# Autodesk Inventor assembly: iDISCO-Sampleholder-Assembly
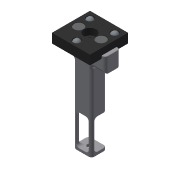
[picture p0: Inventor's stored thumbnail of the model, 180x180]
Saved by Autodesk Inventor 2016 (Build 200138000, 138)
## iProperties
Created: 2019-02-05
Part Number: iDISCO-Sampleholder-Assembly
Document SubType Name: Assembly
Designer: voigt
Author: voigt
## Documents named in this file (3)
- D:\Microscope_Design\CAD_Files\mesoSPIM_design_V4\mesoSPIM_design\mesoSPIM\sample_handling\IDISCO-Sampleholder\iDISCO-Sampleholder-Assembly.iam
- D:\Microscope_Design\CAD_Files\mesoSPIM_design_V4\mesoSPIM_design\library\Thorlabs\kinematic_bases\KBT25_M.ipt
- D:\Microscope_Design\CAD_Files\mesoSPIM_design_V4\mesoSPIM_design\mesoSPIM\sample_handling\IDISCO-Sampleholder\IDISCO-Sampleholder-12mm-60mm_V2_Sascha.ipt
## Components (2 placed, 2 different names)
1. KBT25_M:1 — Mate:1, Angle:1, Mate:2
2. IDISCO-Sampleholder-12mm-60mm_V2_Sascha:1 — Mate:1, Angle:1, Mate:2
## Relationships (3: Mate 2, Angle 1)
- Mate:1: KBT25_M:1 ↔ IDISCO-Sampleholder-12mm-60mm_V2_Sascha:1
- Angle:1 (90 deg): KBT25_M:1 ↔ IDISCO-Sampleholder-12mm-60mm_V2_Sascha:1
- Mate:2: KBT25_M:1 ↔ IDISCO-Sampleholder-12mm-60mm_V2_Sascha:1
